# Autodesk Inventor assembly: CalorimeterAssembly
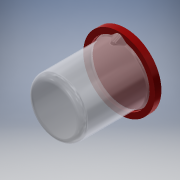
[picture p0: Inventor's stored thumbnail of the model, 180x180]
Saved by Autodesk Inventor 2018 (Build 220112000, 112)
## iProperties
Created: 2020-04-09
Part Number: CalorimeterAssembly
Document SubType Name: Assembly
Designer: Ivan
Author: Ivan
## Documents named in this file (3)
- C:\Users\Ivan\Documents\GitHub\Calorimeter\3D Model\CalorimeterAssembly.iam
- C:\Users\Ivan\Documents\GitHub\Calorimeter\3D Model\CalorimeterCap.ipt
- C:\Users\Ivan\Documents\GitHub\Calorimeter\3D Model\Beaker 2010.ipt
## Components (2 placed, 2 different names)
1. CalorimeterCap:1 — Mate:1, Mate:2
2. Beaker 2010:1 — Mate:1, Mate:2
## Relationships (2: Mate 2)
- Mate:1: CalorimeterCap:1 ↔ Beaker 2010:1
- Mate:2: CalorimeterCap:1 ↔ Beaker 2010:1
